# Autodesk Inventor assembly: 1x6
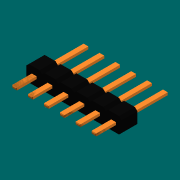
[picture p0: Inventor's stored thumbnail of the model, 180x180]
Saved by Autodesk Inventor 2016 (Build 200138000, 138)
## iProperties
Created: 2014-07-19
Part Number: 1x6
Document SubType Name: Assembly
Designer: Sawaiz Syed
Author: Sawaiz Syed
## Documents named in this file (2)
- C:\Users\Sawaiz\OneDrive\projects\highVoltageMppc\cad\electronics\2.54 Breakaway\1x6.iam
- C:\Users\Sawaiz\OneDrive\projects\highVoltageMppc\cad\electronics\2.54 Breakaway\1x1.iam
## Components (6 placed, 1 different names)
1. 1x1:1 [sub-assembly]
2. 1x1:2 [sub-assembly]
3. 1x1:3 [sub-assembly]
4. 1x1:4 [sub-assembly]
5. 1x1:5 [sub-assembly]
6. 1x1:6 [sub-assembly]
## Component patterns: (6 elements, first: 1x1:1)
